# Autodesk Inventor assembly: Drive W Belly
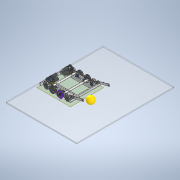
[picture p0: Inventor's stored thumbnail of the model, 180x180]
Saved by Autodesk Inventor 2020 (Build 240168000, 168)
## iProperties
Created: 2020-01-26
Part Number: Drive W Belly
Document SubType Name: Assembly
Designer: aidan
Author: aidan
## Documents named in this file (16)
- C:\Users\aidan\Desktop\T3 Robotics\CAD\Drive W Belly.iam
- C:\Users\aidan\Desktop\T3 Robotics\CAD\Drive Train Actual.iam
- C:\Users\aidan\Desktop\T3 Robotics\CAD\Flat Bar Drive.ipt
- C:\Users\aidan\Desktop\T3 Robotics\CAD\VerseFrame 21in.ipt
- C:\Users\aidan\Desktop\T3 Robotics\CAD\Intake - Piston Mount.ipt
- C:\Users\aidan\Desktop\T3 Robotics\CAD\Intake - Mount.ipt
- C:\Users\aidan\Desktop\T3 Robotics\CAD\Intake - Mount_MIR.ipt
- C:\Users\aidan\Desktop\T3 Robotics\CAD\Intake Basic Piston - Outer.ipt
- C:\Users\aidan\Desktop\T3 Robotics\CAD\Intake Basic Piston - Inner.ipt
- C:\Users\aidan\Desktop\T3 Robotics\CAD\Tony's CAD\FRC Ball.ipt
- C:\Users\aidan\Desktop\T3 Robotics\CAD\Bearing for THUNDER.ipt
- C:\Users\aidan\Desktop\T3 Robotics\CAD\Intake - Side Panel.ipt
- C:\Users\aidan\Desktop\T3 Robotics\CAD\Bearing for THUNDER_MIR.ipt
- C:\Users\aidan\Desktop\T3 Robotics\CAD\Intake - Side Panel_MIR.ipt
- C:\Users\aidan\Desktop\T3 Robotics\CAD\Papa John Connecter.ipt
- C:\Users\aidan\Desktop\T3 Robotics\CAD\GRound.ipt
## Components (26 placed, 15 different names)
1. Drive Train Actual:1 [sub-assembly] — Flush:3, Mate:1, Mate:2, Mate:5, Mate:6, Mate:7, Mate:8, Mate:11, Mate:12, Mate:13, Mate:14, Mate:15, Mate:16, Mate:17, Flush:8
2. Flat Bar Drive:1 — Flush:1, Flush:2, Mate:1, Mate:2
3. Flat Bar Drive:2 — Flush:1, Flush:2, Flush:3, Mate:4, Insert:1, Mate:9, Mate:10, Flush:6
4. VerseFrame 21in:1 — Flush:4, Flush:5, Mate:4, Mate:5, Symmetry:1
5. VerseFrame 21in:2 — Flush:4, Flush:5, Insert:1, Symmetry:1
6. Intake - Piston Mount:1 — Mate:6, Mate:10, Flush:6, Mate:11, Rotational:1
7. Intake - Piston Mount:2 — Mate:7, Mate:8, Mate:9
8. Intake - Mount:2 — Mate:12, Mate:13, Mate:14, Insert:12, Insert:13
9. Intake - Mount_MIR:1 — Mate:15, Mate:16, Mate:17, Insert:10, Insert:11
10. Intake Basic Piston - Outer:1 — Cylindrical:1, Rotational:1, Mate:18
11. Intake Basic Piston - Inner:1 — Cylindrical:1, Mate:18, Rotational:2
12. FRC Ball:1 — Tangent:1
13. Bearing for THUNDER:1 — Insert:13, Insert:17
14. Bearing for THUNDER:2 — Insert:9, Insert:10
15. Bearing for THUNDER:4 — Insert:11
16. Bearing for THUNDER:5 — Insert:12
17. Bearing for THUNDER:6 — Insert:6, Insert:9
18. Bearing for THUNDER:7 — Insert:7
19. Bearing for THUNDER:8 — Insert:8
20. Intake - Side Panel:2 — Insert:6, Insert:7, Insert:8, Flush:7
21. Bearing for THUNDER_MIR:1 — Insert:16, Insert:17
22. Bearing for THUNDER_MIR:2 — Insert:15
23. Bearing for THUNDER_MIR:3 — Insert:14
24. Intake - Side Panel_MIR:1 — Insert:14, Insert:15, Insert:16, Flush:7, Mate:19
25. Papa John Connecter:1 — Rotational:2, Mate:19
26. GRound:1 — Mate:20, Tangent:1
## Relationships (45: Mate 19, Insert 13, Flush 8, RevoluteJoint 2, Symmetry 1, CylindricalJoint 1, Tangent 1)
- Flush:1: Flat Bar Drive:1 ↔ Flat Bar Drive:2
- Flush:2: Flat Bar Drive:1 ↔ Flat Bar Drive:2
- Flush:3: Drive Train Actual:1 ↔ Flat Bar Drive:2
- Mate:1: Drive Train Actual:1 ↔ Flat Bar Drive:1
- Mate:2: Drive Train Actual:1 ↔ Flat Bar Drive:1
- Flush:4: VerseFrame 21in:1 ↔ VerseFrame 21in:2
- Flush:5: VerseFrame 21in:1 ↔ VerseFrame 21in:2
- Mate:4: Flat Bar Drive:2 ↔ VerseFrame 21in:1
- Mate:5: Drive Train Actual:1 ↔ VerseFrame 21in:1
- Insert:1: Flat Bar Drive:2 ↔ VerseFrame 21in:2
- Mate:6: Drive Train Actual:1 ↔ Intake - Piston Mount:1
- Mate:7: Drive Train Actual:1 ↔ Intake - Piston Mount:2
- Mate:8: Drive Train Actual:1 ↔ Intake - Piston Mount:2
- Mate:9: Flat Bar Drive:2 ↔ Intake - Piston Mount:2
- Mate:10: Flat Bar Drive:2 ↔ Intake - Piston Mount:1
- Flush:6: Flat Bar Drive:2 ↔ Intake - Piston Mount:1
- Mate:11: Drive Train Actual:1 ↔ Intake - Piston Mount:1
- Mate:12: Drive Train Actual:1 ↔ Intake - Mount:2
- Mate:13: Drive Train Actual:1 ↔ Intake - Mount:2
- Mate:14: Drive Train Actual:1 ↔ Intake - Mount:2
- Symmetry:1: VerseFrame 21in:1 ↔ VerseFrame 21in:2
- Cylindrical:1: Intake Basic Piston - Outer:1 ↔ Intake Basic Piston - Inner:1
- Rotational:1 [RevoluteJoint] (-0.635 mm): Intake - Piston Mount:1 ↔ Intake Basic Piston - Outer:1
- Insert:6: Bearing for THUNDER:6 ↔ Intake - Side Panel:2
- Insert:7: Bearing for THUNDER:7 ↔ Intake - Side Panel:2
- Insert:8: Bearing for THUNDER:8 ↔ Intake - Side Panel:2
- Insert:9 (6.35 mm): Bearing for THUNDER:2 ↔ Bearing for THUNDER:6
- Mate:15: Drive Train Actual:1 ↔ Intake - Mount_MIR:1
- Mate:16: Drive Train Actual:1 ↔ Intake - Mount_MIR:1
- Mate:17: Drive Train Actual:1 ↔ Intake - Mount_MIR:1
- Insert:10: Intake - Mount_MIR:1 ↔ Bearing for THUNDER:2
- Insert:11: Intake - Mount_MIR:1 ↔ Bearing for THUNDER:4
- Insert:12: Intake - Mount:2 ↔ Bearing for THUNDER:5
- Insert:13: Intake - Mount:2 ↔ Bearing for THUNDER:1
- Insert:14: Bearing for THUNDER_MIR:3 ↔ Intake - Side Panel_MIR:1
- Insert:15: Bearing for THUNDER_MIR:2 ↔ Intake - Side Panel_MIR:1
- Insert:16: Bearing for THUNDER_MIR:1 ↔ Intake - Side Panel_MIR:1
- Insert:17 (12.7 mm): Bearing for THUNDER:1 ↔ Bearing for THUNDER_MIR:1
- Flush:7: Intake - Side Panel:2 ↔ Intake - Side Panel_MIR:1
- Mate:18: Intake Basic Piston - Outer:1 ↔ Intake Basic Piston - Inner:1
- Rotational:2 [RevoluteJoint]: Intake Basic Piston - Inner:1 ↔ Papa John Connecter:1
- Mate:19: Intake - Side Panel_MIR:1 ↔ Papa John Connecter:1
- Flush:8 (52.3875 mm): Drive Train Actual:1
- Mate:20: GRound:1
- Tangent:1: FRC Ball:1 ↔ GRound:1
